# Autodesk Inventor assembly: Assembly
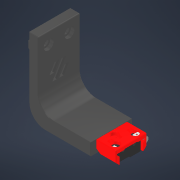
[picture p0: Inventor's stored thumbnail of the model, 180x180]
Saved by Autodesk Inventor 2022.1 (Build 261234000, 234)
## iProperties
Created: 2021-11-02
Part Number: Assembly
Document SubType Name: Assembly
Designer: Rama
Author: Rama
## Documents named in this file (5)
- C:\Users\Rama\Desktop\Glicky\Assembly.iam
- C:\Users\Rama\Desktop\Glicky\Glicky_3D.ipt
- C:\Users\Rama\Desktop\Glicky\Probe.ipt
- C:\Users\Rama\Desktop\Glicky\Dock Mount fixed.ipt
- C:\Users\Rama\Desktop\Glicky\Pin 5x40.ipt
## Components (4 placed, 4 different names)
1. Glicky_3D:1 — Fluchtend:1, Passend:2, Passend:3, Fluchtend:4
2. Probe:1 — Fluchtend:1, Passend:2, Passend:3, Fluchtend:2, Fluchtend:3
3. Dock Mount fixed:1 — Fluchtend:2, Fluchtend:3, Fluchtend:4, Tangential:1, Tangential:2
4. Pin 5x40:1 — Tangential:1, Tangential:2
## Relationships (8: Flush 4, Mate 2, Tangent 2)
- Fluchtend:1 [Flush] (-3.517 mm): Glicky_3D:1 ↔ Probe:1
- Passend:2 [Mate] (-1.5 mm): Glicky_3D:1 ↔ Probe:1
- Passend:3 [Mate]: Glicky_3D:1 ↔ Probe:1
- Fluchtend:2 [Flush] (-0.2 mm): Probe:1 ↔ Dock Mount fixed:1
- Fluchtend:3 [Flush] (-17.225 mm): Probe:1 ↔ Dock Mount fixed:1
- Fluchtend:4 [Flush] (8.1275 mm): Glicky_3D:1 ↔ Dock Mount fixed:1
- Tangential:1 (3.4 mm): Dock Mount fixed:1 ↔ Pin 5x40:1
- Tangential:2 (2 mm): Dock Mount fixed:1 ↔ Pin 5x40:1
